# Autodesk Inventor assembly: wheel_mirrored
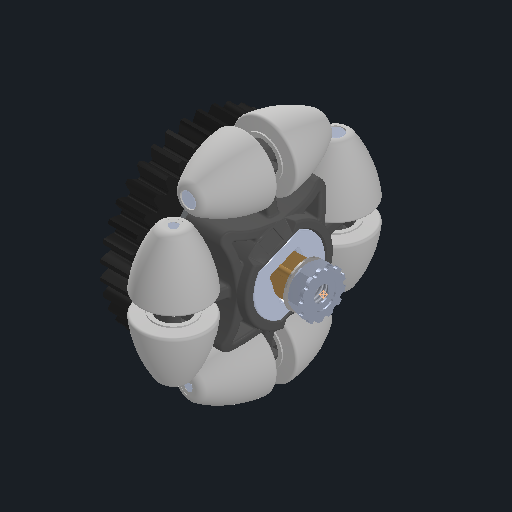
[picture p0: Inventor's stored thumbnail of the model, 512x512]
Saved by Autodesk Inventor 2025 (Build 290162000, 162)
## iProperties
Created: 2024-10-11
Part Number: wheel_mirrored
Document SubType Name: Assembly
Designer: Averey Ku
Author: Averey Ku
## Documents named in this file (7)
- D:\vex_robotics_high_stakes\hardware\cad\bots\high_stakes_v2\chassis_v2\drivebay_mirrored\wheel_mirrored.iam
- D:\vex_robotics_high_stakes\hardware\cad\bots\high_stakes_v2\chassis_v2\drivebay_mirrored\Half Cut HS 36T Gear, No Insert_mirrored.ipt
- D:\vex_robotics_high_stakes\hardware\cad\bots\high_stakes_v2\chassis_v2\drivebay_mirrored\HS Shaft Adapter Circle_mirrored.ipt
- D:\vex_robotics_high_stakes\hardware\cad\bots\high_stakes_v2\chassis_v2\drivebay_mirrored\Nut Keps_mirrored.ipt
- D:\vex_robotics_high_stakes\hardware\cad\robpros_cad_lib\Motion\Spacers\Washer Steel\SWasher .375 OD x .015625.ipt
- D:\vex_robotics_high_stakes\hardware\cad\robpros_cad_lib\Motion\Spacers\Washer Steel.ipt
- D:\vex_robotics_high_stakes\hardware\cad\bots\high_stakes_v2\chassis_v2\drivebay_mirrored\2.00 Omni AS, No Insert_mirrored.ipt
## Components (7 placed, 5 different names)
1. Half Cut HS 36T Gear, No Insert_mirrored:1 — Insert:3, Angle:2, Insert:6, Insert:11
2. HS Shaft Adapter Circle_mirrored:1 — Insert:3, Angle:2, Insert:8
3. Nut Keps_mirrored:1 — Mate:1, Insert:9
4. SWasher .375 OD x .015625:1 — Insert:6
5. 2.00 Omni AS, No Insert_mirrored:1 — Insert:11
6. SWasher .375 OD x .015625:2 — Insert:9, Insert:10
7. HS Shaft Adapter Circle_mirrored:2 — Insert:10, Insert:8
## Relationships (8: Insert 6, Angle 1, Mate 1)
- Insert:3: Half Cut HS 36T Gear, No Insert_mirrored:1 ↔ HS Shaft Adapter Circle_mirrored:1
- Angle:2 (0 deg): Half Cut HS 36T Gear, No Insert_mirrored:1 ↔ HS Shaft Adapter Circle_mirrored:1
- Mate:1: Nut Keps_mirrored:1
- Insert:6: Half Cut HS 36T Gear, No Insert_mirrored:1 ↔ SWasher .375 OD x .015625:1
- Insert:11: Half Cut HS 36T Gear, No Insert_mirrored:1 ↔ 2.00 Omni AS, No Insert_mirrored:1
- Insert:9: Nut Keps_mirrored:1 ↔ SWasher .375 OD x .015625:2
- Insert:10: SWasher .375 OD x .015625:2 ↔ HS Shaft Adapter Circle_mirrored:2
- Insert:8: HS Shaft Adapter Circle_mirrored:1 ↔ HS Shaft Adapter Circle_mirrored:2
